# Autodesk Inventor assembly: Ring Funnel
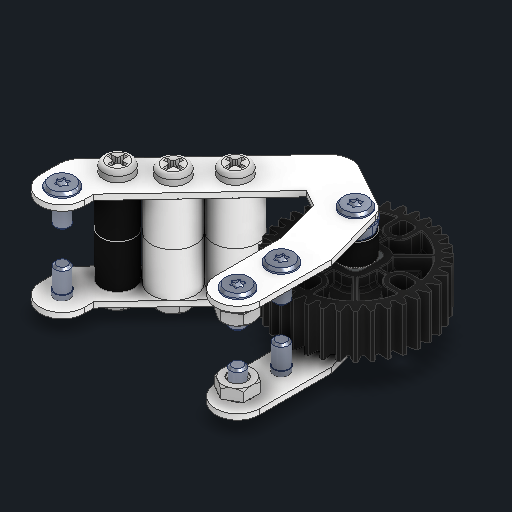
[picture p0: Inventor's stored thumbnail of the model, 512x512]
Saved by Autodesk Inventor 2025.1 (Build 291241000, 241)
## iProperties
Created: 2024-12-17
Part Number: Ring Funnel
Document SubType Name: Assembly
Designer: avere
Author: Averey Ku
## Documents named in this file (18)
- C:\Users\avere\VEX\High Stakes\CAD\V4\Chassis\Drivebay Right\Ring Funnel.iam
- C:\Users\avere\VEX\High Stakes\CAD\V4\Chassis\Drivebay Right\Ring Funnel.ipt
- C:\Users\avere\VEX\High Stakes\CAD\ROBOPROS-CAD-Inventor\Motion\Spacers\Spacer Nylon .375 OD\NSpacer .375 OD x .500.ipt
- C:\Users\avere\VEX\High Stakes\CAD\ROBOPROS-CAD-Inventor\Motion\Spacers\Spacer Nylon .375 OD.ipt
- C:\Users\avere\VEX\High Stakes\CAD\ROBOPROS-CAD-Inventor\Motion\Spacers\Spacer Nylon .500 OD\NSpacer White .500 OD x .500.ipt
- C:\Users\avere\VEX\High Stakes\CAD\ROBOPROS-CAD-Inventor\Motion\Spacers\Spacer Nylon .500 OD.ipt
- C:\Users\avere\VEX\High Stakes\CAD\V4\Chassis\Drivebay Right\HS 36T Gear, No Insert.iam
- C:\Users\avere\VEX\High Stakes\CAD\V4\Chassis\Drivebay Right\NScrew Pan Head Threaded 1.250.ipt
- C:\Users\avere\VEX\High Stakes\CAD\ROBOPROS-CAD-Inventor\Structure\Hardware\Screw Steel - Star\SScrew Star Smooth 1.250.ipt
- C:\Users\avere\VEX\High Stakes\CAD\ROBOPROS-CAD-Inventor\Structure\Hardware\Screw Steel - Star.ipt
- C:\Users\avere\VEX\High Stakes\CAD\V4\Chassis\Drivebay Right\Nut Nylon Thread-Forming.ipt
- C:\Users\avere\VEX\High Stakes\CAD\ROBOPROS-CAD-Inventor\Structure\Hardware\Screw Shoulder Robosource\SScrew Shoulder Smooth .375 x .12.ipt
- C:\Users\avere\VEX\High Stakes\CAD\ROBOPROS-CAD-Inventor\Structure\Hardware\Screw Shoulder Robosource.ipt
- C:\Users\avere\VEX\High Stakes\CAD\ROBOPROS-CAD-Inventor\Motion\Spacers\Washer Steel\SWasher .375 OD x .062500.ipt
- C:\Users\avere\VEX\High Stakes\CAD\ROBOPROS-CAD-Inventor\Motion\Spacers\Washer Steel.ipt
- C:\Users\avere\VEX\High Stakes\CAD\ROBOPROS-CAD-Inventor\Motion\Spacers\Washer Steel\SWasher .375 OD x .031250.ipt
- C:\Users\avere\VEX\High Stakes\CAD\V4\Chassis\Drivebay Right\Nut Keps.ipt
- C:\Users\avere\VEX\High Stakes\CAD\ROBOPROS-CAD-Inventor\Motion\Spacers\Spacer Nylon .375 OD\NSpacer .375 OD x .250.ipt
## Components (30 placed, 12 different names)
1. Ring Funnel:1 — Mate:1, Insert:1, Insert:3, Insert:5, Insert:10, Insert:9, Insert:11, Insert:12, Insert:19, Insert:17, Insert:18, Insert:23, Insert:27
2. Ring Funnel:2 — Mate:1, Insert:1, Insert:6, Insert:8, Insert:13, Insert:14, Insert:15, Insert:16, Insert:21, Insert:20, Insert:22, Insert:24, Insert:26
3. NSpacer .375 OD x .500:1 — Insert:2
4. NSpacer .375 OD x .500:2 — Insert:3, Insert:2
5. NSpacer White .500 OD x .500:1 — Insert:4
6. NSpacer White .500 OD x .500:2 — Insert:5, Insert:4
7. HS 36T Gear, No Insert:1 [sub-assembly] — Insert:6
8. NSpacer White .500 OD x .500:3 — Insert:8, Insert:7
9. NSpacer White .500 OD x .500:4 — Insert:7
10. NScrew Pan Head Threaded 1.250:1 — Insert:10
11. NScrew Pan Head Threaded 1.250:2 — Insert:9
12. SScrew Star Smooth 1.250:1 — Insert:11
13. NScrew Pan Head Threaded 1.250:3 — Insert:12
14. Nut Nylon Thread-Forming:1 — Insert:13
15. Nut Nylon Thread-Forming:2 — Insert:14
16. Nut Nylon Thread-Forming:3 — Insert:15
17. Nut Nylon Thread-Forming:4 — Insert:16
18. SScrew Shoulder Smooth .375 x .12:1 — Insert:19
19. SScrew Shoulder Smooth .375 x .12:2 — Insert:17
20. SScrew Shoulder Smooth .375 x .12:3 — Insert:18
21. SScrew Shoulder Smooth .375 x .12:4 — Insert:21
22. SScrew Shoulder Smooth .375 x .12:5 — Insert:20
23. SScrew Shoulder Smooth .375 x .12:6 — Insert:22
24. Nut Nylon Thread-Forming:5 — Insert:23
25. Nut Nylon Thread-Forming:6 — Insert:24
26. SWasher .375 OD x .062500:1 — Insert:26, Insert:25
27. SWasher .375 OD x .031250:2 — Insert:25
28. Nut Keps:1 — Insert:27, Insert:29
29. SWasher .375 OD x .062500:3 — Insert:28
30. NSpacer .375 OD x .250:3 — Insert:29, Insert:28
## Relationships (30: Insert 29, Mate 1)
- Mate:1: Ring Funnel:1 ↔ Ring Funnel:2
- Insert:1 (25.4 mm): Ring Funnel:1 ↔ Ring Funnel:2
- Insert:3: Ring Funnel:1 ↔ NSpacer .375 OD x .500:2
- Insert:2: NSpacer .375 OD x .500:1 ↔ NSpacer .375 OD x .500:2
- Insert:5: Ring Funnel:1 ↔ NSpacer White .500 OD x .500:2
- Insert:4: NSpacer White .500 OD x .500:1 ↔ NSpacer White .500 OD x .500:2
- Insert:6 (2.3813 mm): Ring Funnel:2 ↔ HS 36T Gear, No Insert:1
- Insert:8: Ring Funnel:2 ↔ NSpacer White .500 OD x .500:3
- Insert:7: NSpacer White .500 OD x .500:3 ↔ NSpacer White .500 OD x .500:4
- Insert:10: Ring Funnel:1 ↔ NScrew Pan Head Threaded 1.250:1
- Insert:9: Ring Funnel:1 ↔ NScrew Pan Head Threaded 1.250:2
- Insert:11: Ring Funnel:1 ↔ SScrew Star Smooth 1.250:1
- Insert:12: Ring Funnel:1 ↔ NScrew Pan Head Threaded 1.250:3
- Insert:13: Ring Funnel:2 ↔ Nut Nylon Thread-Forming:1
- Insert:14: Ring Funnel:2 ↔ Nut Nylon Thread-Forming:2
- Insert:15: Ring Funnel:2 ↔ Nut Nylon Thread-Forming:3
- Insert:16: Ring Funnel:2 ↔ Nut Nylon Thread-Forming:4
- Insert:19: Ring Funnel:1 ↔ SScrew Shoulder Smooth .375 x .12:1
- Insert:17: Ring Funnel:1 ↔ SScrew Shoulder Smooth .375 x .12:2
- Insert:18: Ring Funnel:1 ↔ SScrew Shoulder Smooth .375 x .12:3
- Insert:21: Ring Funnel:2 ↔ SScrew Shoulder Smooth .375 x .12:4
- Insert:20: Ring Funnel:2 ↔ SScrew Shoulder Smooth .375 x .12:5
- Insert:22: Ring Funnel:2 ↔ SScrew Shoulder Smooth .375 x .12:6
- Insert:23 (1.5875 mm): Ring Funnel:1 ↔ Nut Nylon Thread-Forming:5
- Insert:24 (1.5875 mm): Ring Funnel:2 ↔ Nut Nylon Thread-Forming:6
- Insert:26: Ring Funnel:2 ↔ SWasher .375 OD x .062500:1
- Insert:25: SWasher .375 OD x .062500:1 ↔ SWasher .375 OD x .031250:2
- Insert:27: Ring Funnel:1 ↔ Nut Keps:1
- Insert:29: Nut Keps:1 ↔ NSpacer .375 OD x .250:3
- Insert:28: SWasher .375 OD x .062500:3 ↔ NSpacer .375 OD x .250:3
